# Autodesk Inventor assembly: Arm_Right
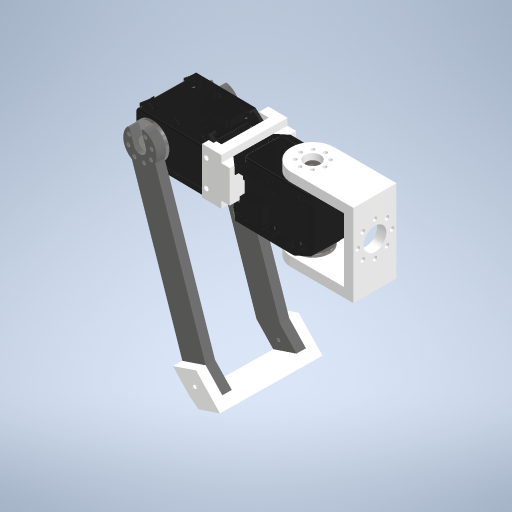
[picture p0: Inventor's stored thumbnail of the model, 512x512]
Saved by Autodesk Inventor 2024.3 (Build 283343000, 343)
## iProperties
Created: 2024-09-18
Part Number: Arm_Right
Document SubType Name: Assembly
Designer: 구지현
Author: 구지현
## Documents named in this file (8)
- C:\Users\구지현\Desktop\19th_intern_kdy_fight_robot\부품\Upper_Body\Arm\Arm_Right.iam
- C:\Users\구지현\Desktop\19th_intern_kdy_fight_robot\부품\Upper_Body\Arm\Hand.ipt
- C:\Users\구지현\Desktop\19th_intern_kdy_fight_robot\부품\Upper_Body\Arm\Hand_Connection_Parts.ipt
- C:\Users\구지현\Desktop\19th_intern_kdy_fight_robot\부품\Upper_Body\Arm\Middle_Arm_Fixing_Parts.ipt
- C:\Users\구지현\Desktop\19th_intern_kdy_fight_robot\부품\Upper_Body\Arm\28Horn.ipt
- C:\Users\구지현\Desktop\19th_intern_kdy_fight_robot\부품\Upper_Body\Arm\Shoulder_Fixing_Parts_Left_MIR.ipt
- C:\Users\구지현\Desktop\19th_intern_kdy_fight_robot\부품\ROBOTIS(Inventor 2024 ver.)\다이나믹셀\MX-28T_R+idle.ipt.iam
- MX-28T_R+idle.ipt
## Components (8 placed, 6 different names)
1. Hand:1 — 메이트:5, 메이트:6, 플러쉬:2, 삽입:8
2. Hand_Connection_Parts:1 — 플러쉬:2, 삽입:8
3. Middle_Arm_Fixing_Parts:1 — 메이트:7, 메이트:8, 메이트:9, 메이트:10
4. 28Horn:2 — 메이트:5, 메이트:6, 삽입:11
5. Shoulder_Fixing_Parts_Left_MIR:1 — 플러쉬:1, 삽입:9
6. 28Horn:3 — 삽입:9, 삽입:10
7. MX-28T_R+idle.ipt:1 [sub-assembly] — 삽입:11, 메이트:9, 메이트:10
8. MX-28T_R+idle.ipt:2 [sub-assembly] — 삽입:10, 메이트:7, 메이트:8
## Relationships (12: Mate 6, Insert 4, Flush 2)
- 플러쉬:1 [Flush]: Shoulder_Fixing_Parts_Left_MIR:1
- 메이트:5 [Mate]: Hand:1 ↔ 28Horn:2
- 메이트:6 [Mate]: Hand:1 ↔ 28Horn:2
- 플러쉬:2 [Flush]: Hand:1 ↔ Hand_Connection_Parts:1
- 삽입:8 [Insert]: Hand:1 ↔ Hand_Connection_Parts:1
- 삽입:9 [Insert]: Shoulder_Fixing_Parts_Left_MIR:1 ↔ 28Horn:3
- 삽입:10 [Insert]: 28Horn:3 ↔ MX-28T_R+idle.ipt:2
- 메이트:7 [Mate]: Middle_Arm_Fixing_Parts:1 ↔ MX-28T_R+idle.ipt:2
- 메이트:8 [Mate]: Middle_Arm_Fixing_Parts:1 ↔ MX-28T_R+idle.ipt:2
- 삽입:11 [Insert]: 28Horn:2 ↔ MX-28T_R+idle.ipt:1
- 메이트:9 [Mate]: Middle_Arm_Fixing_Parts:1 ↔ MX-28T_R+idle.ipt:1
- 메이트:10 [Mate]: Middle_Arm_Fixing_Parts:1 ↔ MX-28T_R+idle.ipt:1
